# Autodesk Inventor assembly: 2924-1015-1000 assembly
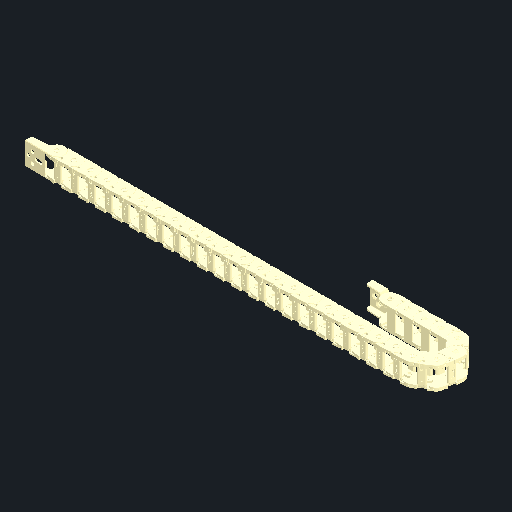
[picture p0: Inventor's stored thumbnail of the model, 512x512]
Saved by Autodesk Inventor 2026.2 (Build 302298000, 298)
## iProperties
Created: 2023-10-18
Part Number: 2924-1015-1000 assembly
Description: STEP AP203
Document SubType Name: Assembly
Designer: Kenji
Sending System: SolidWorks 2016
Preprocessor: SwSTEP 2.0
Title: 2924-1015-1000 assembly.STEP
Revision Number: ANY
## Documents named in this file (4)
- C:\Users\Kenji\Documents\GitHub\DiyCNC-\COTS-Parts\10x15-CarbleCarrierXAxis-2924-1015-1000.iam
- C:\Users\Kenji\Downloads\2924-1015-1000\2924-1015-1000 assembly\2924-1015-1000 assembly\2924-1015 End 1.ipt
- C:\Users\Kenji\Downloads\2924-1015-1000\2924-1015-1000 assembly\2924-1015-1000 assembly\2924-1015 link.ipt
- C:\Users\Kenji\Downloads\2924-1015-1000\2924-1015-1000 assembly\2924-1015-1000 assembly\2924-1015 End 2.ipt
## Components (30 placed, 10 different names)
1. 2924-1015 End 1_1 — Mate:2, Angle:1, Mate:33, Angle:2
2. 2924-1015 link_2 — Mate:2, Mate:4, Mate:5, Mate:6, Mate:24, Mate:25, Mate:26
3. 2924-1015 link_3 — Mate:10, Mate:11, Mate:12, Mate:13, Mate:14
4. 2924-1015 link_4 — Mate:4, Mate:5, Mate:6, Mate:7, Mate:8, Mate:9
5. 2924-1015 link_5 — Mate:7, Mate:8, Mate:9, Mate:10, Mate:11, Mate:12
6. 2924-1015 link_6 — Mate:13, Mate:14, Angle:1, Mate:15, Mate:16, Mate:17
7. 2924-1015 link_7 — Mate:15, Mate:16, Mate:17, Mate:18, Mate:19, Mate:20
8. 2924-1015 End 2:2 — Mate:22, Mate:23, Tangent:1
9. 2924-1015 link:76 — Mate:24, Mate:25, Mate:26, Mate:27, Mate:28, Mate:29
10. 2924-1015 link:77 — Mate:27, Mate:28, Mate:29, Mate:30, Mate:31, Mate:32
11. 2924-1015 link:78 — Mate:30, Mate:31, Mate:32, Mate:33, Angle:2
12. 2924-1015 link_8 — Mate:18, Mate:19, Mate:20
13. 2924-1015 link:58
14. 2924-1015 link:59
15. 2924-1015 link:60
16. 2924-1015 link:61
17. 2924-1015 link:62
18. 2924-1015 link:63
19. 2924-1015 link:64
20. 2924-1015 link:65
21. 2924-1015 link:66
22. 2924-1015 link:67
23. 2924-1015 link:68
24. 2924-1015 link:69
25. 2924-1015 link:70
26. 2924-1015 link:71
27. 2924-1015 link:72
28. 2924-1015 link:73
29. 2924-1015 link:74 — Mate:22
30. 2924-1015 link:75 — Mate:23, Tangent:1
## Component patterns: (19 elements, first: 2924-1015 link_8)
## Relationships (33: Mate 30, Angle 2, Tangent 1)
- Mate:2: 2924-1015 End 1_1 ↔ 2924-1015 link_2
- Mate:4: 2924-1015 link_2 ↔ 2924-1015 link_4
- Mate:5: 2924-1015 link_2 ↔ 2924-1015 link_4
- Mate:6: 2924-1015 link_2 ↔ 2924-1015 link_4
- Mate:7: 2924-1015 link_4 ↔ 2924-1015 link_5
- Mate:8: 2924-1015 link_4 ↔ 2924-1015 link_5
- Mate:9: 2924-1015 link_4 ↔ 2924-1015 link_5
- Mate:10: 2924-1015 link_3 ↔ 2924-1015 link_5
- Mate:11: 2924-1015 link_3 ↔ 2924-1015 link_5
- Mate:12: 2924-1015 link_3 ↔ 2924-1015 link_5
- Mate:13: 2924-1015 link_3 ↔ 2924-1015 link_6
- Mate:14: 2924-1015 link_3 ↔ 2924-1015 link_6
- Angle:1 (0 deg): 2924-1015 End 1_1 ↔ 2924-1015 link_6
- Mate:15: 2924-1015 link_6 ↔ 2924-1015 link_7
- Mate:16: 2924-1015 link_6 ↔ 2924-1015 link_7
- Mate:17: 2924-1015 link_6 ↔ 2924-1015 link_7
- Mate:18: 2924-1015 link_7 ↔ 2924-1015 link_8
- Mate:19: 2924-1015 link_7 ↔ 2924-1015 link_8
- Mate:20: 2924-1015 link_7 ↔ 2924-1015 link_8
- Mate:22: 2924-1015 End 2:2 ↔ 2924-1015 link:74
- Mate:23: 2924-1015 End 2:2 ↔ 2924-1015 link:75
- Tangent:1: 2924-1015 End 2:2 ↔ 2924-1015 link:75
- Mate:24: 2924-1015 link_2 ↔ 2924-1015 link:76
- Mate:25: 2924-1015 link_2 ↔ 2924-1015 link:76
- Mate:26: 2924-1015 link_2 ↔ 2924-1015 link:76
- Mate:27: 2924-1015 link:76 ↔ 2924-1015 link:77
- Mate:28: 2924-1015 link:76 ↔ 2924-1015 link:77
- Mate:29: 2924-1015 link:76 ↔ 2924-1015 link:77
- Mate:30: 2924-1015 link:77 ↔ 2924-1015 link:78
- Mate:31: 2924-1015 link:77 ↔ 2924-1015 link:78
- Mate:32: 2924-1015 link:77 ↔ 2924-1015 link:78
- Mate:33: 2924-1015 End 1_1 ↔ 2924-1015 link:78
- Angle:2 (0 deg): 2924-1015 End 1_1 ↔ 2924-1015 link:78
